# Autodesk Inventor assembly: ASY MSC 002 отстойник осветлитель
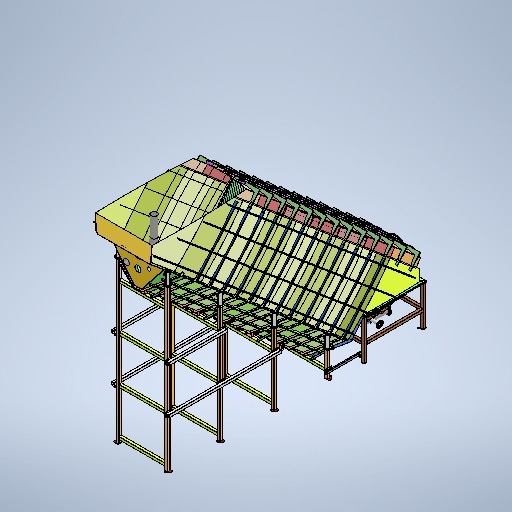
[picture p0: Inventor's stored thumbnail of the model, 512x512]
Saved by Autodesk Inventor 2025 (Build 290162010, 162A)
## iProperties
Created: 2024-09-05
Part Number: ASY MSC 002 отстойник осветлитель
Document SubType Name: Assembly
Designer: admin
Mass: 2.83156e+06 g
Surface Area: 4.02448e+06 cm^2
Volume: 367916 cm^3
Density: 7.69621 g/cm^3
Author: admin
## Documents named in this file (36)
- C:\Users\pokla\Documents\Inventor\Отстойник осветлитель\Manturovo_Se-clar-Gleb\ASY MSC 002 отстойник осветлитель.iam
- C:\Users\pokla\Documents\Inventor\Отстойник осветлитель\Manturovo_Se-clar-Gleb\ASY MSC 900.1 base frame.iam
- C:\Users\pokla\Documents\Inventor\Отстойник осветлитель\Manturovo_Se-clar-Gleb\ASY MSC 100 cone.iam
- C:\Users\pokla\Documents\Inventor\Отстойник осветлитель\Manturovo_Se-clar-Gleb\MSC 401 sheet lowerback.ipt
- C:\Users\pokla\Documents\Inventor\Отстойник осветлитель\Manturovo_Se-clar-Gleb\MSC 701 face 1.ipt
- C:\Users\pokla\Documents\Inventor\Отстойник осветлитель\Manturovo_Se-clar-Gleb\MSC 705 ridge 3.ipt
- C:\Users\pokla\Documents\Inventor\Отстойник осветлитель\Manturovo_Se-clar-Gleb\MSC 713 tube.ipt
- C:\Users\pokla\Documents\Inventor\Отстойник осветлитель\Manturovo_Se-clar-Gleb\ISO 5251 Bends 3D without straight ends(90 deg) DN150 11 11.ipt
- C:\Users\pokla\Documents\Inventor\Отстойник осветлитель\Manturovo_Se-clar-Gleb\MSC 408 stringer lowerback.ipt
- C:\Users\pokla\Documents\Inventor\Отстойник осветлитель\Manturovo_Se-clar-Gleb\MSC 703 face 2.ipt
- C:\Users\pokla\Documents\Inventor\Отстойник осветлитель\Manturovo_Se-clar-Gleb\MSC 702 face 3.ipt
- C:\Users\pokla\Documents\Inventor\Отстойник осветлитель\Manturovo_Se-clar-Gleb\MSC 704 face 4.ipt
- C:\Users\pokla\Documents\Inventor\Отстойник осветлитель\Manturovo_Se-clar-Gleb\ASY MSC 900.3 base frame.iam
- C:\Users\pokla\Documents\Inventor\Отстойник осветлитель\Manturovo_Se-clar-Gleb\Pillars\ASY MSC 900.5 base frame.iam
- C:\Users\pokla\Documents\Inventor\Отстойник осветлитель\Manturovo_Se-clar-Gleb\Pillars\ASY MSC 900.4  base frame.iam
- C:\Users\pokla\Documents\Inventor\Отстойник осветлитель\Manturovo_Se-clar-Gleb\Pillars\ASY MSC 900.6 base frame.iam
- C:\Users\pokla\Documents\Inventor\Отстойник осветлитель\Manturovo_Se-clar-Gleb\ASY MSC 200 BACK.iam
- C:\Users\pokla\Documents\Inventor\Отстойник осветлитель\Manturovo_Se-clar-Gleb\ASY MSC 300.2 LEFT BOARD.iam
- C:\Users\pokla\Documents\Inventor\Отстойник осветлитель\Manturovo_Se-clar-Gleb\ASY MSC 300.1 RIGHT BOARD.iam
- C:\Users\pokla\Documents\Inventor\Отстойник осветлитель\Manturovo_Se-clar-Gleb\ASY MSC 500 BELLY.iam
- C:\Users\pokla\Documents\Inventor\Отстойник осветлитель\Manturovo_Se-clar-Gleb\ASY MSC 900.2 support.iam
- C:\Users\pokla\Documents\Inventor\Отстойник осветлитель\Manturovo_Se-clar-Gleb\ASY MSC 600 cone exit back.iam
- C:\Users\pokla\Documents\Inventor\Отстойник осветлитель\Manturovo_Se-clar-Gleb\ASY MSC 800 gills.iam
- C:\Users\pokla\Documents\Inventor\Отстойник осветлитель\Manturovo_Se-clar-Gleb\ASY MSC 400 Accsess hatch.iam
- C:\Users\pokla\Documents\Inventor\Отстойник осветлитель\Manturovo_Se-clar-Gleb\MSC DIM 000 settler-clarifier.ipt
- C:\Users\pokla\Documents\Inventor\Отстойник осветлитель\Manturovo_Se-clar-Gleb\MSC DIM 001 frame.ipt
- C:\Users\pokla\Documents\Inventor\Отстойник осветлитель\Manturovo_Se-clar-Gleb\ASY MSC 900.7 base frame transverse.iam
- C:\Users\pokla\Documents\Inventor\Отстойник осветлитель\Manturovo_Se-clar-Gleb\ASY MSC 900.8 base frame transverse.iam
- C:\Users\pokla\Documents\Inventor\Отстойник осветлитель\Manturovo_Se-clar-Gleb\MSC 908 transverse pillar plate.ipt
- C:\Users\pokla\Documents\Inventor\Отстойник осветлитель\Manturovo_Se-clar-Gleb\Part2.ipt
- C:\Users\pokla\Documents\Inventor\Отстойник осветлитель\Manturovo_Se-clar-Gleb\MSC 900.9 base frame transverse.ipt
- C:\Users\pokla\Documents\Inventor\Отстойник осветлитель\Manturovo_Se-clar-Gleb\ASY MSC 700 water tray.iam
- C:\Users\pokla\Documents\Inventor\Отстойник осветлитель\Manturovo_Se-clar-Gleb\ASY 940 linkage.iam
- C:\Users\pokla\Documents\Inventor\Отстойник осветлитель\Manturovo_Se-clar-Gleb\Part1.ipt
- C:\Users\pokla\Documents\Inventor\Отстойник осветлитель\Manturovo_Se-clar-Gleb\Part3.ipt
- C:\Users\pokla\Documents\Inventor\Отстойник осветлитель\Manturovo_Se-clar-Gleb\Part4.ipt
## Components (51 placed, 35 different names)
1. MSC DIM 000 settler-clarifier:1
2. MSC DIM 001 frame:1
3. MSC 401 sheet lowerback:1 — Mate:29, Mate:30, Mate:31
4. MSC 705 ridge 3:1
5. MSC 704 face 4:1
6. ASY MSC 300.2 LEFT BOARD:1 [sub-assembly] — Rigid:11, Mate:34
7. ASY MSC 300.1 RIGHT BOARD:1 [sub-assembly] — Rigid:10, Flush:17
8. ASY MSC 700 water tray:1 [sub-assembly]
9. MSC 908 transverse pillar plate:4 — Mate:50, Flush:16, Flush:18
10. MSC 908 transverse pillar plate:8
11. ASY MSC 100 cone:1 [sub-assembly] — Mate:19, Flush:6, Mate:29, Rigid:17
12. ASY MSC 900.1 base frame:1 [sub-assembly] — Flush:4, Mate:18, Flush:5, Mate:19, Mate:44, Mate:47, Mate:50, Flush:16
13. ASY MSC 400 Accsess hatch:1 [sub-assembly]
14. MSC 408 stringer lowerback:2
15. MSC 408 stringer lowerback:1
16. ASY MSC 900.2 support:7 [sub-assembly]
17. ASY MSC 900.2 support:3 [sub-assembly] — Cylindrical:4, Mate:25
18. ASY MSC 600 cone exit back:1 [sub-assembly] — Rigid:17
19. ASY MSC 900.3 base frame:1 [sub-assembly] — Mate:23, Mate:24, Cylindrical:4, Mate:44, Mate:45, Rigid:31, Rigid:32, Rigid:33
20. ASY 940 linkage:2 [sub-assembly] — Rigid:31
21. ASY 940 linkage:1 [sub-assembly] — Rigid:32, Flush:18
22. ASY MSC 900.8 base frame transverse:1 [sub-assembly] — Rigid:21
23. ASY MSC 900.8 base frame transverse:2 [sub-assembly] — Rigid:22
24. Part1:1 — Rigid:33, Mate:68, Mate:69, Mate:70
25. MSC 900.9 base frame transverse:5 — Mate:68, Mate:69, Mate:70
26. Part2:2 — Rigid:27, Mate:59, Mate:67
27. MSC 900.9 base frame transverse:2 — Mate:59, Mate:67
28. Part3:1 — Rigid:34, Mate:71, Mate:72, Mate:73
29. MSC 900.9 base frame transverse:6 — Mate:71, Mate:72, Mate:73
30. Part4:1 — Rigid:35, Mate:74, Mate:75, Mate:76
31. MSC 900.9 base frame transverse:4 — Mate:74, Mate:75, Mate:76
32. ASY MSC 900.2 support:5 [sub-assembly]
33. ASY MSC 900.2 support:2 [sub-assembly]
34. ASY MSC 900.7 base frame transverse:2 [sub-assembly] — Rigid:20
35. ASY MSC 900.7 base frame transverse:1 [sub-assembly] — Rigid:19
36. ASY MSC 900.4  base frame:1 [sub-assembly] — Mate:32, Mate:33, Mate:45, Mate:46, Rigid:27
37. ASY MSC 200 BACK:1 [sub-assembly] — Flush:8, Mate:31
38. ASY MSC 900.2 support:6 [sub-assembly] — Cylindrical:7, Mate:41
39. ASY MSC 900.2 support:1 [sub-assembly] — Cylindrical:8, Mate:40
40. ASY MSC 900.2 support:8 [sub-assembly] — Cylindrical:5, Mate:43
41. ASY MSC 900.2 support:4 [sub-assembly] — Cylindrical:6, Mate:42
42. MSC 702 face 3:1 — Mate:34, Mate:35, Mate:36, Mate:66
43. MSC 703 face 2:1 — Flush:13, Flush:17, Mate:66
44. MSC 713 tube:2
45. ISO 5251 Bends 3D without straight ends(90 deg) DN150 11:1
46. MSC 713 tube:1 — Rigid:4
47. MSC 701 face 1:1 — Rigid:4, Flush:9, Mate:35
48. ASY MSC 500 BELLY:1 [sub-assembly] — Flush:7, Mate:22, Mate:25, Rigid:10, Rigid:11, Mate:40, Mate:41, Mate:42, Mate:43
49. ASY MSC 900.5 base frame:1 [sub-assembly] — Flush:11, Cylindrical:7, Cylindrical:8, Mate:46, Mate:48, Rigid:34
50. ASY MSC 900.6 base frame:1 [sub-assembly] — Mate:38, Mate:39, Cylindrical:5, Cylindrical:6, Mate:47, Rigid:19, Rigid:20, Rigid:21, Rigid:22, Rigid:35
51. ASY MSC 800 gills:1 [sub-assembly] — Mate:22
## Relationships (92: Mate 50, WeldJoint 19, Flush 14, CylindricalJoint 8, RevoluteJoint 1)
- [Mate]: MSC 401 sheet lowerback:1 ↔ ASY MSC 100 cone:1
- [WeldJoint]: ISO 5251 Bends 3D without straight ends(90 deg) DN150 11:1 ↔ MSC 713 tube:1
- [Mate]: ASY MSC 100 cone:1 ↔ MSC 408 stringer lowerback:1
- [RevoluteJoint]: MSC 713 tube:2 ↔ ISO 5251 Bends 3D without straight ends(90 deg) DN150 11:1
- Rigid:4 [WeldJoint]: MSC 713 tube:1 ↔ MSC 701 face 1:1
- [Mate]: ASY MSC 100 cone:1 ↔ MSC 408 stringer lowerback:2
- [Mate]: ASY MSC 600 cone exit back:1 ↔ ASY MSC 500 BELLY:1
- [Flush]: ASY MSC 100 cone:1 ↔ ASY MSC 900.1 base frame:1
- [WeldJoint]: MSC 705 ridge 3:1 ↔ ASY MSC 700 water tray:1
- [WeldJoint]: MSC 705 ridge 3:1 ↔ ASY MSC 700 water tray:1
- [Flush]: ASY MSC 600 cone exit back:1 ↔ ASY MSC 500 BELLY:1
- [Mate]: ASY MSC 500 BELLY:1 ↔ ASY MSC 800 gills:1
- [Mate]: MSC 701 face 1:1 ↔ ASY MSC 500 BELLY:1
- [Mate] (-5 mm): MSC 701 face 1:1 ↔ ASY MSC 500 BELLY:1
- [Mate] (3 mm): ASY MSC 900.2 support:2 ↔ ASY MSC 500 BELLY:1
- [Mate] (3 mm): ASY MSC 900.2 support:5 ↔ ASY MSC 500 BELLY:1
- [Mate] (3 mm): ASY MSC 900.2 support:7 ↔ ASY MSC 500 BELLY:1
- [CylindricalJoint]: ASY MSC 900.2 support:5 ↔ ASY MSC 900.4  base frame:1
- [CylindricalJoint]: ASY MSC 900.2 support:2 ↔ ASY MSC 900.4  base frame:1
- [Mate] (-2860 mm): ASY MSC 200 BACK:1 ↔ ASY MSC 500 BELLY:1
- [CylindricalJoint]: ASY MSC 900.2 support:7 ↔ ASY MSC 900.3 base frame:1
- [Flush]: ASY MSC 900.3 base frame:1 ↔ ASY MSC 900.4  base frame:1
- Flush:4: ASY MSC 900.1 base frame:1
- Mate:18 (4 mm): ASY MSC 900.1 base frame:1
- Flush:5: ASY MSC 900.1 base frame:1
- Mate:19: ASY MSC 100 cone:1 ↔ ASY MSC 900.1 base frame:1
- Flush:6: ASY MSC 100 cone:1
- Flush:7: ASY MSC 500 BELLY:1
- Flush:8: ASY MSC 200 BACK:1
- Mate:22: ASY MSC 500 BELLY:1 ↔ ASY MSC 800 gills:1
- Mate:23: ASY MSC 900.3 base frame:1
- Mate:24: ASY MSC 900.3 base frame:1
- Cylindrical:4: ASY MSC 900.2 support:3 ↔ ASY MSC 900.3 base frame:1
- Mate:25 (3 mm): ASY MSC 900.2 support:3 ↔ ASY MSC 500 BELLY:1
- Flush:9: MSC 701 face 1:1
- Mate:29: MSC 401 sheet lowerback:1 ↔ ASY MSC 100 cone:1
- Mate:30: MSC 401 sheet lowerback:1
- Mate:31: MSC 401 sheet lowerback:1 ↔ ASY MSC 200 BACK:1
- Rigid:10 [WeldJoint] (-25 mm): ASY MSC 300.1 RIGHT BOARD:1 ↔ ASY MSC 500 BELLY:1
- Rigid:11 [WeldJoint] (-25 mm): ASY MSC 300.2 LEFT BOARD:1 ↔ ASY MSC 500 BELLY:1
- Flush:11: ASY MSC 900.5 base frame:1
- Mate:32: ASY MSC 900.4  base frame:1
- Mate:33: ASY MSC 900.4  base frame:1
- Mate:34: ASY MSC 300.2 LEFT BOARD:1 ↔ MSC 702 face 3:1
- Mate:35: MSC 702 face 3:1 ↔ MSC 701 face 1:1
- [WeldJoint]: MSC 705 ridge 3:1 ↔ ASY MSC 700 water tray:1
- Mate:36: MSC 702 face 3:1
- Mate:38: ASY MSC 900.6 base frame:1
- Mate:39: ASY MSC 900.6 base frame:1
- Cylindrical:5: ASY MSC 900.2 support:8 ↔ ASY MSC 900.6 base frame:1
- Cylindrical:6: ASY MSC 900.2 support:4 ↔ ASY MSC 900.6 base frame:1
- Cylindrical:7: ASY MSC 900.2 support:6 ↔ ASY MSC 900.5 base frame:1
- Cylindrical:8: ASY MSC 900.2 support:1 ↔ ASY MSC 900.5 base frame:1
- Mate:40 (3 mm): ASY MSC 900.2 support:1 ↔ ASY MSC 500 BELLY:1
- Mate:41 (3 mm): ASY MSC 900.2 support:6 ↔ ASY MSC 500 BELLY:1
- Mate:42 (3 mm): ASY MSC 900.2 support:4 ↔ ASY MSC 500 BELLY:1
- Mate:43 (3 mm): ASY MSC 900.2 support:8 ↔ ASY MSC 500 BELLY:1
- Flush:13: MSC 703 face 2:1
- Mate:44 (820 mm): ASY MSC 900.1 base frame:1 ↔ ASY MSC 900.3 base frame:1
- Mate:45 (1430 mm): ASY MSC 900.3 base frame:1 ↔ ASY MSC 900.4  base frame:1
- Mate:46 (1430 mm): ASY MSC 900.4  base frame:1 ↔ ASY MSC 900.5 base frame:1
- Mate:47 (5315 mm): ASY MSC 900.1 base frame:1 ↔ ASY MSC 900.6 base frame:1
- Rigid:17 [WeldJoint]: ASY MSC 100 cone:1 ↔ ASY MSC 600 cone exit back:1
- Mate:48: ASY MSC 900.5 base frame:1
- Rigid:19 [WeldJoint]: ASY MSC 900.7 base frame transverse:1 ↔ ASY MSC 900.6 base frame:1
- Rigid:20 [WeldJoint]: ASY MSC 900.7 base frame transverse:2 ↔ ASY MSC 900.6 base frame:1
- Rigid:21 [WeldJoint]: ASY MSC 900.8 base frame transverse:1 ↔ ASY MSC 900.6 base frame:1
- Rigid:22 [WeldJoint]: ASY MSC 900.8 base frame transverse:2 ↔ ASY MSC 900.6 base frame:1
- Mate:50: MSC 908 transverse pillar plate:4 ↔ ASY MSC 900.1 base frame:1
- [Mate]: Part2:2 ↔ MSC 900.9 base frame transverse:2
- Rigid:27 [WeldJoint]: Part2:2 ↔ ASY MSC 900.4  base frame:1
- Mate:59: Part2:2 ↔ MSC 900.9 base frame transverse:2
- Flush:16 (-40 mm): MSC 908 transverse pillar plate:4 ↔ ASY MSC 900.1 base frame:1
- Flush:17: ASY MSC 300.1 RIGHT BOARD:1 ↔ MSC 703 face 2:1
- Mate:66: MSC 702 face 3:1 ↔ MSC 703 face 2:1
- [WeldJoint]: MSC 908 transverse pillar plate:8 ↔ ASY 940 linkage:2
- Rigid:31 [WeldJoint]: ASY MSC 900.3 base frame:1 ↔ ASY 940 linkage:2
- Rigid:32 [WeldJoint]: ASY MSC 900.3 base frame:1 ↔ ASY 940 linkage:1
- Flush:18: MSC 908 transverse pillar plate:4 ↔ ASY 940 linkage:1
- Mate:67 (11 mm): Part2:2 ↔ MSC 900.9 base frame transverse:2
- Rigid:33 [WeldJoint]: ASY MSC 900.3 base frame:1 ↔ Part1:1
- Mate:68: Part1:1 ↔ MSC 900.9 base frame transverse:5
- Mate:69 (11 mm): Part1:1 ↔ MSC 900.9 base frame transverse:5
- Mate:70: Part1:1 ↔ MSC 900.9 base frame transverse:5
- Rigid:34 [WeldJoint]: Part3:1 ↔ ASY MSC 900.5 base frame:1
- Mate:71: Part3:1 ↔ MSC 900.9 base frame transverse:6
- Mate:72 (11 mm): Part3:1 ↔ MSC 900.9 base frame transverse:6
- Mate:73: Part3:1 ↔ MSC 900.9 base frame transverse:6
- Rigid:35 [WeldJoint]: Part4:1 ↔ ASY MSC 900.6 base frame:1
- Mate:74: Part4:1 ↔ MSC 900.9 base frame transverse:4
- Mate:75 (11 mm): Part4:1 ↔ MSC 900.9 base frame transverse:4
- Mate:76: Part4:1 ↔ MSC 900.9 base frame transverse:4
## Named parameters: d131_d129 = 0 mm, d334_d122 = 0 mm
